# Autodesk Inventor assembly: NASA-20
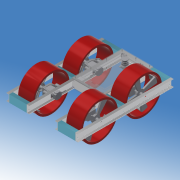
[picture p0: Inventor's stored thumbnail of the model, 180x180]
Saved by Autodesk Inventor 2020 (Build 240168000, 168)
## iProperties
RuleStatus: InUse
Created: 2019-09-05
Part Number: NASA-20
Document SubType Name: Assembly
Designer: Rick Szalay
Author: Rick Szalay
## Documents named in this file (22)
- C:\Users\mpark\Documents\NASA20\Inventor Files\NASA-20\NASA-20\NASA-20.iam
- C:\Users\mpark\Documents\NASA20\Inventor Files\NASA-20\NASA-20\A428.ipt
- C:\Users\mpark\Documents\NASA20\Inventor Files\NASA-20\NASA-20\NASA-20-WH-01.ipt
- C:\Users\mpark\Documents\NASA20\Inventor Files\NASA-20\NASA-20\NASA-20-WT-01.ipt
- C:\Users\mpark\Documents\NASA20\Inventor Files\NASA-20\NASA-20\FR\NASA-20-FR.iam
- C:\Users\mpark\Documents\NASA20\Inventor Files\NASA-20\NASA-20\FR\NASA-20-TB-01.ipt
- C:\Users\mpark\Documents\NASA20\Inventor Files\NASA-20\NASA-20\FR\NASA-20-OP-01.ipt
- C:\Users\mpark\Documents\NASA20\Inventor Files\NASA-20\NASA-20\FR\NASA-20-MP-01.ipt
- C:\Users\Matt\Documents\Inventor\Content Center Files\R2020\en-US\ANSI B18.2.1(3)\ANSI B18.2.1 - 1_4-20 UNC - 5.5(3).ipt
- C:\Users\Matt\Documents\Inventor\Content Center Files\R2020\en-US\ANSI B18.2.2(09)\ANSI B18.2.2 - 1_4 - 20(2).ipt
- C:\Users\mpark\Documents\NASA20\Inventor Files\NASA-20\NASA-20\Tube Replacements.iam
- C:\Users\mpark\Documents\NASA20\Inventor Files\NASA-20\NASA-20\E-Box\NASA-20-EBOX-B-01.ipt
- NASA-20-EBOX-B-01.ipt
- C:\Users\mpark\Documents\NASA20\Inventor Files\NASA-20\NASA-20\E-Box\NASA-20-EBOX-T-01.ipt
- NASA-20-EBOX-T-01.ipt
- C:\Users\mpark\Documents\NASA20\Inventor Files\NASA-20\NASA-20\E-Box\NASA-20-EBOX-T2-01.ipt
- C:\Users\mpark\Documents\NASA20\Inventor Files\NASA-20\NASA-20\E-Box\NASA-20-EBOX-LID-01.ipt
- C:\Users\mpark\Documents\NASA20\Inventor Files\NASA-20\NASA-20\E-Box\1603A230_UNFINISHED BRASS SURFACE-MNT HINGE W HOLES.ipt
- C:\Users\mpark\OneDrive\Documents\Inventor\Content Center Files\R2020\en-US\ANSI B18.2.4.2M\ANSI B18.2.4.2M - M3x0.5 - 5.5.ipt
- C:\Users\mpark\OneDrive\Documents\Inventor\Content Center Files\R2020\en-US\AS 1420\AS 1420 - 1973 - M3 x 14.ipt
- C:\Users\mpark\OneDrive\Documents\Inventor\Content Center Files\R2020\en-US\AS 1420\AS 1420 - 1973 - M3 x 16.ipt
- C:\Users\mpark\Documents\NASA20\Inventor Files\NASA-20\NASA-20\E-Box\9235K200_METAL 30 MM PANEL-MOUNT SWITCH.ipt
## Components (104 placed, 19 different names)
1. A428:1 — Mate:38, Mate:39, Flush:28, Mate:41
2. NASA-20-WH-01:1 — Mate:6, Flush:9, Mate:40, Mate:41
3. NASA-20-WT-01:1 — Mate:6, Flush:9, Mate:61, Tangent:1
4. NASA-20-FR:1 [sub-assembly] — Mate:20, Mate:21, Flush:13, Mate:22, Mate:23, Mate:24, Mate:25, Mate:26, Mate:27, Mate:28, Mate:29, Mate:30, Mate:31, Mate:32, Mate:33, Mate:34, Mate:35, Flush:26, Flush:27, Flush:29, Mate:42, Mate:58, Flush:36, Mate:59, Mate:60, Flush:37, Flush:38, Insert:13, Insert:14, Insert:15, Insert:16, Insert:17, Insert:18, Insert:19, Insert:20, Insert:21, Insert:22, Insert:23, Insert:24, Mate:64, Mate:65, Mate:66, Mate:67, Mate:68, Mate:69, Mate:70, Mate:71, Mate:72, Mate:73, Mate:74, Mate:75, Mate:76, Mate:77, Mate:78, Mate:79, Mate:80, Mate:81, Mate:82, Mate:83, Flush:39, Flush:40, Flush:41, Flush:42, Flush:51
5. NASA-20-OP-01:1 — Flush:24, Flush:25, Mate:37, Flush:26, Flush:27, Mate:63, Insert:7, Insert:8, Insert:9, Insert:10, Insert:11, Insert:12
6. NASA-20-OP-01:2 — Flush:24, Flush:25, Mate:36, Insert:1, Insert:2, Insert:3, Insert:4, Insert:5, Insert:6
7. NASA-20-MP-01:1 — Mate:38, Mate:39, Flush:28, Mate:40, Flush:29, Mate:42
8. A428:2
9. NASA-20-WH-01:2
10. NASA-20-WT-01:2 — Mate:62, Tangent:1
11. NASA-20-MP-01:2 — Mate:58, Flush:36
12. A428:3
13. NASA-20-WH-01:3
14. NASA-20-WT-01:3 — Mate:62, Mate:63
15. NASA-20-MP-01:3 — Mate:59, Flush:37
16. A428:4
17. NASA-20-WH-01:4
18. NASA-20-WT-01:4 — Mate:61
19. NASA-20-MP-01:4 — Mate:60, Flush:38
20. 9235K200_METAL 30 MM PANEL-MOUNT SWITCH:1
21. NASA-20-TB-01:1 — Flush:14, Mate:22, Mate:23
22. NASA-20-TB-01:2 — Flush:14, Flush:15, Mate:24, Mate:36
23. NASA-20-TB-01:3 — Flush:15, Flush:16, Mate:25
24. NASA-20-TB-01:4 — Flush:16, Flush:17, Mate:26
25. NASA-20-TB-01:5 — Flush:17, Flush:18, Mate:27
26. NASA-20-TB-01:6 — Flush:18, Mate:28
27. NASA-20-TB-01:7 — Mate:34, Mate:37
28. NASA-20-TB-01:8 — Mate:35
29. NASA-20-TB-01:9 — Mate:30
30. NASA-20-TB-01:10 — Mate:33
31. NASA-20-TB-01:11 — Mate:32
32. NASA-20-TB-01:12 — Mate:29, Mate:31
33. AS 1420 - Metric M3 x 16:11 — Insert:39
34. AS 1420 - Metric M3 x 16:12 — Insert:40
35. AS 1420 - Metric M3 x 16:13 — Insert:41
36. AS 1420 - Metric M3 x 16:14 — Insert:42
37. AS 1420 - Metric M3 x 16:15 — Insert:43
38. AS 1420 - Metric M3 x 16:16 — Insert:44
39. AS 1420 - Metric M3 x 16:17 — Insert:45
40. AS 1420 - Metric M3 x 16:18 — Insert:46
41. AS 1420 - Metric M3 x 16:19 — Insert:47
42. AS 1420 - Metric M3 x 16:20 — Insert:48
43. AS 1420 - Metric M3 x 16:1 — Insert:29
44. AS 1420 - Metric M3 x 16:2 — Insert:30
45. AS 1420 - Metric M3 x 16:3 — Insert:31
46. AS 1420 - Metric M3 x 16:4 — Insert:32
47. AS 1420 - Metric M3 x 16:5 — Insert:33
48. AS 1420 - Metric M3 x 16:6 — Insert:34
49. AS 1420 - Metric M3 x 16:7 — Insert:35
50. AS 1420 - Metric M3 x 16:8 — Insert:36
51. AS 1420 - Metric M3 x 16:9 — Insert:37
52. AS 1420 - Metric M3 x 16:10 — Insert:38
53. ANSI B18.2.4.2M M3x0.5:3 — Mate:104, Mate:106
54. ANSI B18.2.4.2M M3x0.5:4 — Mate:107, Mate:108
55. ANSI B18.2.4.2M M3x0.5:5 — Mate:109, Mate:110
56. ANSI B18.2.4.2M M3x0.5:6 — Mate:111, Mate:112
57. ANSI B18.2.4.2M M3x0.5:7 — Mate:113, Mate:114
58. ANSI B18.2.4.2M M3x0.5:8 — Mate:115, Mate:116
59. ANSI B18.2.4.2M M3x0.5:9 — Mate:117, Mate:118
60. AS 1420 - Metric M3 x 14:5 — Mate:98, Mate:99, Mate:117
61. AS 1420 - Metric M3 x 14:6 — Mate:100, Mate:101, Mate:115
62. AS 1420 - Metric M3 x 14:7 — Insert:27, Mate:111
63. AS 1420 - Metric M3 x 14:8 — Insert:28, Mate:113
64. AS 1420 - Metric M3 x 14:1 — Insert:25, Mate:109
65. AS 1420 - Metric M3 x 14:2 — Insert:26, Mate:97
66. AS 1420 - Metric M3 x 14:3 — Mate:92, Mate:96, Mate:107
67. AS 1420 - Metric M3 x 14:4 — Mate:94, Mate:95, Mate:104
68. ANSI B18.2.4.2M M3x0.5:1 — Mate:97, Mate:105
69. Hex Cap Screw - Inch 1/4-20 UNC - 5.5:13 — Insert:1
70. Hex Cap Screw - Inch 1/4-20 UNC - 5.5:14 — Insert:2
71. Hex Cap Screw - Inch 1/4-20 UNC - 5.5:15 — Insert:3
72. Hex Cap Screw - Inch 1/4-20 UNC - 5.5:16 — Insert:4
73. Hex Cap Screw - Inch 1/4-20 UNC - 5.5:17 — Insert:5
74. Hex Cap Screw - Inch 1/4-20 UNC - 5.5:18 — Insert:6
75. Hex Cap Screw - Inch 1/4-20 UNC - 5.5:20 — Insert:7
76. Hex Cap Screw - Inch 1/4-20 UNC - 5.5:19 — Insert:8
77. Hex Cap Screw - Inch 1/4-20 UNC - 5.5:21 — Insert:9
78. Hex Cap Screw - Inch 1/4-20 UNC - 5.5:22 — Insert:10
79. Hex Cap Screw - Inch 1/4-20 UNC - 5.5:23 — Insert:11
80. Hex Cap Screw - Inch 1/4-20 UNC - 5.5:24 — Insert:12
81. Hex Nut - Inch 1/4 - 20:13 — Insert:13
82. Hex Nut - Inch 1/4 - 20:14 — Insert:14
83. Hex Nut - Inch 1/4 - 20:15 — Insert:15
84. Hex Nut - Inch 1/4 - 20:16 — Insert:16
85. Hex Nut - Inch 1/4 - 20:17 — Insert:17
86. Hex Nut - Inch 1/4 - 20:18 — Insert:18
87. Hex Nut - Inch 1/4 - 20:19 — Insert:19
88. Hex Nut - Inch 1/4 - 20:20 — Insert:20
89. Hex Nut - Inch 1/4 - 20:21 — Insert:21
90. Hex Nut - Inch 1/4 - 20:22 — Insert:22
91. Hex Nut - Inch 1/4 - 20:23 — Insert:23
92. Hex Nut - Inch 1/4 - 20:24 — Insert:24
93. Tube Replacements:1 [sub-assembly] — Mate:64, Mate:70, Mate:81
94. Tube Replacements:2 [sub-assembly] — Mate:65, Mate:72, Mate:80
95. Tube Replacements:3 [sub-assembly] — Mate:66, Mate:71, Mate:79
96. Tube Replacements:4 [sub-assembly] — Mate:69, Mate:75, Mate:76
97. Tube Replacements:5 [sub-assembly] — Mate:68, Mate:74, Mate:77
98. Tube Replacements:6 [sub-assembly] — Mate:67, Mate:73, Mate:78
99. 1603A230_UNFINISHED BRASS SURFACE-MNT HINGE W HOLES:1 — Mate:90, Flush:49, Insert:25, Insert:26, Mate:92, Mate:94, Mate:95, Mate:96, Flush:50, Flush:51
100. 1603A230_UNFINISHED BRASS SURFACE-MNT HINGE W HOLES:2 — Mate:91, Flush:48, Mate:98, Mate:99, Mate:100, Mate:101, Insert:27, Insert:28, Flush:50
101. NASA-20-EBOX-LID-01:1 — Mate:85, Flush:45, Mate:86, Mate:87
102. NASA-20-EBOX-T2-01:2 — Mate:84, Flush:43, Flush:44, Flush:45, Mate:86, Mate:87, Mate:90, Mate:91, Flush:48, Flush:49, Insert:29, Insert:30, Insert:31, Insert:32, Insert:33, Insert:34, Insert:35, Insert:36, Insert:37, Insert:38
103. NASA-20-EBOX-T-01:1 — Mate:83, Flush:41, Flush:42, Mate:84, Flush:43, Flush:44, Mate:85, Mate:105, Mate:106, Mate:108, Mate:110, Mate:112, Mate:114, Mate:116, Mate:118
104. NASA-20-EBOX-B-01:1 — Mate:82, Flush:39, Flush:40, Insert:39, Insert:40, Insert:41, Insert:42, Insert:43, Insert:44, Insert:45, Insert:46, Insert:47, Insert:48
## Relationships (182: Mate 95, Insert 48, Flush 38, Tangent 1)
- Mate:6: NASA-20-WH-01:1 ↔ NASA-20-WT-01:1
- Flush:9 (19.05 mm): NASA-20-WH-01:1 ↔ NASA-20-WT-01:1
- Mate:20: NASA-20-FR:1
- Mate:21: NASA-20-FR:1
- Flush:13: NASA-20-FR:1
- Flush:14: NASA-20-TB-01:1 ↔ NASA-20-TB-01:2
- Flush:15: NASA-20-TB-01:2 ↔ NASA-20-TB-01:3
- Flush:16: NASA-20-TB-01:3 ↔ NASA-20-TB-01:4
- Flush:17: NASA-20-TB-01:4 ↔ NASA-20-TB-01:5
- Flush:18: NASA-20-TB-01:5 ↔ NASA-20-TB-01:6
- Mate:22: NASA-20-FR:1 ↔ NASA-20-TB-01:1
- Mate:23: NASA-20-FR:1 ↔ NASA-20-TB-01:1
- Mate:24: NASA-20-FR:1 ↔ NASA-20-TB-01:2
- Mate:25: NASA-20-FR:1 ↔ NASA-20-TB-01:3
- Mate:26: NASA-20-FR:1 ↔ NASA-20-TB-01:4
- Mate:27: NASA-20-FR:1 ↔ NASA-20-TB-01:5
- Mate:28: NASA-20-FR:1 ↔ NASA-20-TB-01:6
- [Flush]: NASA-20-TB-01:7 ↔ NASA-20-TB-01:8
- [Flush]: NASA-20-TB-01:8 ↔ NASA-20-TB-01:9
- [Flush]: NASA-20-TB-01:9 ↔ NASA-20-TB-01:10
- [Flush]: NASA-20-TB-01:10 ↔ NASA-20-TB-01:11
- [Flush]: NASA-20-TB-01:11 ↔ NASA-20-TB-01:12
- Mate:29: NASA-20-FR:1 ↔ NASA-20-TB-01:12
- Mate:30: NASA-20-FR:1 ↔ NASA-20-TB-01:9
- Mate:31: NASA-20-FR:1 ↔ NASA-20-TB-01:12
- Mate:32: NASA-20-FR:1 ↔ NASA-20-TB-01:11
- Mate:33: NASA-20-FR:1 ↔ NASA-20-TB-01:10
- Mate:34: NASA-20-FR:1 ↔ NASA-20-TB-01:7
- Mate:35: NASA-20-FR:1 ↔ NASA-20-TB-01:8
- Flush:24: NASA-20-OP-01:1 ↔ NASA-20-OP-01:2
- Flush:25: NASA-20-OP-01:1 ↔ NASA-20-OP-01:2
- Mate:36: NASA-20-OP-01:2 ↔ NASA-20-TB-01:2
- Mate:37: NASA-20-OP-01:1 ↔ NASA-20-TB-01:7
- Flush:26: NASA-20-FR:1 ↔ NASA-20-OP-01:1
- Flush:27: NASA-20-FR:1 ↔ NASA-20-OP-01:1
- Mate:38: A428:1 ↔ NASA-20-MP-01:1
- Mate:39: A428:1 ↔ NASA-20-MP-01:1
- Flush:28: A428:1 ↔ NASA-20-MP-01:1
- Mate:40 (1.5875 mm): NASA-20-WH-01:1 ↔ NASA-20-MP-01:1
- Mate:41: A428:1 ↔ NASA-20-WH-01:1
- Flush:29: NASA-20-FR:1 ↔ NASA-20-MP-01:1
- Mate:42: NASA-20-FR:1 ↔ NASA-20-MP-01:1
- [Mate]: NASA-20-WH-01:2 ↔ NASA-20-WT-01:2
- [Flush] (19.05 mm): NASA-20-WH-01:2 ↔ NASA-20-WT-01:2
- [Mate]: A428:2 ↔ NASA-20-MP-01:2
- [Mate]: A428:2 ↔ NASA-20-MP-01:2
- [Flush]: A428:2 ↔ NASA-20-MP-01:2
- [Mate] (1.5875 mm): NASA-20-WH-01:2 ↔ NASA-20-MP-01:2
- [Mate]: A428:2 ↔ NASA-20-WH-01:2
- [Mate]: NASA-20-WH-01:3 ↔ NASA-20-WT-01:3
- [Flush] (19.05 mm): NASA-20-WH-01:3 ↔ NASA-20-WT-01:3
- [Mate]: A428:3 ↔ NASA-20-MP-01:3
- [Mate]: A428:3 ↔ NASA-20-MP-01:3
- [Flush]: A428:3 ↔ NASA-20-MP-01:3
- [Mate] (1.5875 mm): NASA-20-WH-01:3 ↔ NASA-20-MP-01:3
- [Mate]: A428:3 ↔ NASA-20-WH-01:3
- [Mate]: NASA-20-WH-01:4 ↔ NASA-20-WT-01:4
- [Flush] (19.05 mm): NASA-20-WH-01:4 ↔ NASA-20-WT-01:4
- [Mate]: A428:4 ↔ NASA-20-MP-01:4
- [Mate]: A428:4 ↔ NASA-20-MP-01:4
- [Flush]: A428:4 ↔ NASA-20-MP-01:4
- [Mate] (1.5875 mm): NASA-20-WH-01:4 ↔ NASA-20-MP-01:4
- [Mate]: A428:4 ↔ NASA-20-WH-01:4
- Mate:58: NASA-20-FR:1 ↔ NASA-20-MP-01:2
- Flush:36: NASA-20-FR:1 ↔ NASA-20-MP-01:2
- Mate:59: NASA-20-FR:1 ↔ NASA-20-MP-01:3
- Mate:60: NASA-20-FR:1 ↔ NASA-20-MP-01:4
- Flush:37: NASA-20-FR:1 ↔ NASA-20-MP-01:3
- Flush:38: NASA-20-FR:1 ↔ NASA-20-MP-01:4
- Mate:61: NASA-20-WT-01:1 ↔ NASA-20-WT-01:4
- Mate:62: NASA-20-WT-01:2 ↔ NASA-20-WT-01:3
- Tangent:1 (50.8 mm): NASA-20-WT-01:1 ↔ NASA-20-WT-01:2
- Mate:63: NASA-20-OP-01:1 ↔ NASA-20-WT-01:3
- Insert:1: NASA-20-OP-01:2 ↔ Hex Cap Screw - Inch 1/4-20 UNC - 5.5:13
- Insert:2: NASA-20-OP-01:2 ↔ Hex Cap Screw - Inch 1/4-20 UNC - 5.5:14
- Insert:3: NASA-20-OP-01:2 ↔ Hex Cap Screw - Inch 1/4-20 UNC - 5.5:15
- Insert:4: NASA-20-OP-01:2 ↔ Hex Cap Screw - Inch 1/4-20 UNC - 5.5:16
- Insert:5: NASA-20-OP-01:2 ↔ Hex Cap Screw - Inch 1/4-20 UNC - 5.5:17
- Insert:6: NASA-20-OP-01:2 ↔ Hex Cap Screw - Inch 1/4-20 UNC - 5.5:18
- Insert:7: NASA-20-OP-01:1 ↔ Hex Cap Screw - Inch 1/4-20 UNC - 5.5:20
- Insert:8: NASA-20-OP-01:1 ↔ Hex Cap Screw - Inch 1/4-20 UNC - 5.5:19
- Insert:9: NASA-20-OP-01:1 ↔ Hex Cap Screw - Inch 1/4-20 UNC - 5.5:21
- Insert:10: NASA-20-OP-01:1 ↔ Hex Cap Screw - Inch 1/4-20 UNC - 5.5:22
- Insert:11: NASA-20-OP-01:1 ↔ Hex Cap Screw - Inch 1/4-20 UNC - 5.5:23
- Insert:12: NASA-20-OP-01:1 ↔ Hex Cap Screw - Inch 1/4-20 UNC - 5.5:24
- Insert:13: NASA-20-FR:1 ↔ Hex Nut - Inch 1/4 - 20:13
- Insert:14: NASA-20-FR:1 ↔ Hex Nut - Inch 1/4 - 20:14
- Insert:15: NASA-20-FR:1 ↔ Hex Nut - Inch 1/4 - 20:15
- Insert:16: NASA-20-FR:1 ↔ Hex Nut - Inch 1/4 - 20:16
- Insert:17: NASA-20-FR:1 ↔ Hex Nut - Inch 1/4 - 20:17
- Insert:18: NASA-20-FR:1 ↔ Hex Nut - Inch 1/4 - 20:18
- Insert:19: NASA-20-FR:1 ↔ Hex Nut - Inch 1/4 - 20:19
- Insert:20: NASA-20-FR:1 ↔ Hex Nut - Inch 1/4 - 20:20
- Insert:21: NASA-20-FR:1 ↔ Hex Nut - Inch 1/4 - 20:21
- Insert:22: NASA-20-FR:1 ↔ Hex Nut - Inch 1/4 - 20:22
- Insert:23: NASA-20-FR:1 ↔ Hex Nut - Inch 1/4 - 20:23
- Insert:24: NASA-20-FR:1 ↔ Hex Nut - Inch 1/4 - 20:24
- Mate:64: NASA-20-FR:1 ↔ Tube Replacements:1
- Mate:65: NASA-20-FR:1 ↔ Tube Replacements:2
- Mate:66: NASA-20-FR:1 ↔ Tube Replacements:3
- Mate:67: NASA-20-FR:1 ↔ Tube Replacements:6
- Mate:68: NASA-20-FR:1 ↔ Tube Replacements:5
- Mate:69: NASA-20-FR:1 ↔ Tube Replacements:4
- Mate:70: NASA-20-FR:1 ↔ Tube Replacements:1
- Mate:71: NASA-20-FR:1 ↔ Tube Replacements:3
- Mate:72: NASA-20-FR:1 ↔ Tube Replacements:2
- Mate:73: NASA-20-FR:1 ↔ Tube Replacements:6
- Mate:74: NASA-20-FR:1 ↔ Tube Replacements:5
- Mate:75: NASA-20-FR:1 ↔ Tube Replacements:4
- Mate:76: NASA-20-FR:1 ↔ Tube Replacements:4
- Mate:77: NASA-20-FR:1 ↔ Tube Replacements:5
- Mate:78: NASA-20-FR:1 ↔ Tube Replacements:6
- Mate:79: NASA-20-FR:1 ↔ Tube Replacements:3
- Mate:80: NASA-20-FR:1 ↔ Tube Replacements:2
- Mate:81: NASA-20-FR:1 ↔ Tube Replacements:1
- Mate:82: NASA-20-FR:1 ↔ NASA-20-EBOX-B-01:1
- Mate:83: NASA-20-FR:1 ↔ NASA-20-EBOX-T-01:1
- Flush:39: NASA-20-FR:1 ↔ NASA-20-EBOX-B-01:1
- Flush:40: NASA-20-FR:1 ↔ NASA-20-EBOX-B-01:1
- Flush:41: NASA-20-FR:1 ↔ NASA-20-EBOX-T-01:1
- Flush:42: NASA-20-FR:1 ↔ NASA-20-EBOX-T-01:1
- Mate:84: NASA-20-EBOX-T2-01:2 ↔ NASA-20-EBOX-T-01:1
- Flush:43: NASA-20-EBOX-T2-01:2 ↔ NASA-20-EBOX-T-01:1
- Flush:44: NASA-20-EBOX-T2-01:2 ↔ NASA-20-EBOX-T-01:1
- Mate:85: NASA-20-EBOX-LID-01:1 ↔ NASA-20-EBOX-T-01:1
- Flush:45: NASA-20-EBOX-LID-01:1 ↔ NASA-20-EBOX-T2-01:2
- Mate:86 (1 mm): NASA-20-EBOX-LID-01:1 ↔ NASA-20-EBOX-T2-01:2
- Mate:87 (1 mm): NASA-20-EBOX-LID-01:1 ↔ NASA-20-EBOX-T2-01:2
- Mate:90: 1603A230_UNFINISHED BRASS SURFACE-MNT HINGE W HOLES:1 ↔ NASA-20-EBOX-T2-01:2
- Mate:91: 1603A230_UNFINISHED BRASS SURFACE-MNT HINGE W HOLES:2 ↔ NASA-20-EBOX-T2-01:2
- Flush:48 (38.1 mm): 1603A230_UNFINISHED BRASS SURFACE-MNT HINGE W HOLES:2 ↔ NASA-20-EBOX-T2-01:2
- Flush:49 (38.1 mm): 1603A230_UNFINISHED BRASS SURFACE-MNT HINGE W HOLES:1 ↔ NASA-20-EBOX-T2-01:2
- Insert:25: AS 1420 - Metric M3 x 14:1 ↔ 1603A230_UNFINISHED BRASS SURFACE-MNT HINGE W HOLES:1
- Insert:26: AS 1420 - Metric M3 x 14:2 ↔ 1603A230_UNFINISHED BRASS SURFACE-MNT HINGE W HOLES:1
- Mate:92: AS 1420 - Metric M3 x 14:3 ↔ 1603A230_UNFINISHED BRASS SURFACE-MNT HINGE W HOLES:1
- Mate:94: AS 1420 - Metric M3 x 14:4 ↔ 1603A230_UNFINISHED BRASS SURFACE-MNT HINGE W HOLES:1
- Mate:95: AS 1420 - Metric M3 x 14:4 ↔ 1603A230_UNFINISHED BRASS SURFACE-MNT HINGE W HOLES:1
- Mate:96: AS 1420 - Metric M3 x 14:3 ↔ 1603A230_UNFINISHED BRASS SURFACE-MNT HINGE W HOLES:1
- Mate:97: AS 1420 - Metric M3 x 14:2 ↔ ANSI B18.2.4.2M M3x0.5:1
- Mate:98: AS 1420 - Metric M3 x 14:5 ↔ 1603A230_UNFINISHED BRASS SURFACE-MNT HINGE W HOLES:2
- Mate:99: AS 1420 - Metric M3 x 14:5 ↔ 1603A230_UNFINISHED BRASS SURFACE-MNT HINGE W HOLES:2
- Mate:100: AS 1420 - Metric M3 x 14:6 ↔ 1603A230_UNFINISHED BRASS SURFACE-MNT HINGE W HOLES:2
- Mate:101: AS 1420 - Metric M3 x 14:6 ↔ 1603A230_UNFINISHED BRASS SURFACE-MNT HINGE W HOLES:2
- Insert:27: AS 1420 - Metric M3 x 14:7 ↔ 1603A230_UNFINISHED BRASS SURFACE-MNT HINGE W HOLES:2
- Insert:28: AS 1420 - Metric M3 x 14:8 ↔ 1603A230_UNFINISHED BRASS SURFACE-MNT HINGE W HOLES:2
- Flush:50: 1603A230_UNFINISHED BRASS SURFACE-MNT HINGE W HOLES:1 ↔ 1603A230_UNFINISHED BRASS SURFACE-MNT HINGE W HOLES:2
- Flush:51 (25.4 mm): NASA-20-FR:1 ↔ 1603A230_UNFINISHED BRASS SURFACE-MNT HINGE W HOLES:1
- Mate:104: ANSI B18.2.4.2M M3x0.5:3 ↔ AS 1420 - Metric M3 x 14:4
- Mate:105 (-3.175 mm): ANSI B18.2.4.2M M3x0.5:1 ↔ NASA-20-EBOX-T-01:1
- Mate:106: ANSI B18.2.4.2M M3x0.5:3 ↔ NASA-20-EBOX-T-01:1
- Mate:107: ANSI B18.2.4.2M M3x0.5:4 ↔ AS 1420 - Metric M3 x 14:3
- Mate:108: ANSI B18.2.4.2M M3x0.5:4 ↔ NASA-20-EBOX-T-01:1
- Mate:109: ANSI B18.2.4.2M M3x0.5:5 ↔ AS 1420 - Metric M3 x 14:1
- Mate:110: ANSI B18.2.4.2M M3x0.5:5 ↔ NASA-20-EBOX-T-01:1
- Mate:111: ANSI B18.2.4.2M M3x0.5:6 ↔ AS 1420 - Metric M3 x 14:7
- Mate:112: ANSI B18.2.4.2M M3x0.5:6 ↔ NASA-20-EBOX-T-01:1
- Mate:113: ANSI B18.2.4.2M M3x0.5:7 ↔ AS 1420 - Metric M3 x 14:8
- Mate:114: ANSI B18.2.4.2M M3x0.5:7 ↔ NASA-20-EBOX-T-01:1
- Mate:115: ANSI B18.2.4.2M M3x0.5:8 ↔ AS 1420 - Metric M3 x 14:6
- Mate:116 (-3.175 mm): ANSI B18.2.4.2M M3x0.5:8 ↔ NASA-20-EBOX-T-01:1
- Mate:117: ANSI B18.2.4.2M M3x0.5:9 ↔ AS 1420 - Metric M3 x 14:5
- Mate:118 (-3.175 mm): ANSI B18.2.4.2M M3x0.5:9 ↔ NASA-20-EBOX-T-01:1
- Insert:29: AS 1420 - Metric M3 x 16:1 ↔ NASA-20-EBOX-T2-01:2
- Insert:30: AS 1420 - Metric M3 x 16:2 ↔ NASA-20-EBOX-T2-01:2
- Insert:31: AS 1420 - Metric M3 x 16:3 ↔ NASA-20-EBOX-T2-01:2
- Insert:32: AS 1420 - Metric M3 x 16:4 ↔ NASA-20-EBOX-T2-01:2
- Insert:33: AS 1420 - Metric M3 x 16:5 ↔ NASA-20-EBOX-T2-01:2
- Insert:34: AS 1420 - Metric M3 x 16:6 ↔ NASA-20-EBOX-T2-01:2
- Insert:35: AS 1420 - Metric M3 x 16:7 ↔ NASA-20-EBOX-T2-01:2
- Insert:36: AS 1420 - Metric M3 x 16:8 ↔ NASA-20-EBOX-T2-01:2
- Insert:37: AS 1420 - Metric M3 x 16:9 ↔ NASA-20-EBOX-T2-01:2
- Insert:38: AS 1420 - Metric M3 x 16:10 ↔ NASA-20-EBOX-T2-01:2
- Insert:39: AS 1420 - Metric M3 x 16:11 ↔ NASA-20-EBOX-B-01:1
- Insert:40: AS 1420 - Metric M3 x 16:12 ↔ NASA-20-EBOX-B-01:1
- Insert:41: AS 1420 - Metric M3 x 16:13 ↔ NASA-20-EBOX-B-01:1
- Insert:42: AS 1420 - Metric M3 x 16:14 ↔ NASA-20-EBOX-B-01:1
- Insert:43: AS 1420 - Metric M3 x 16:15 ↔ NASA-20-EBOX-B-01:1
- Insert:44: AS 1420 - Metric M3 x 16:16 ↔ NASA-20-EBOX-B-01:1
- Insert:45: AS 1420 - Metric M3 x 16:17 ↔ NASA-20-EBOX-B-01:1
- Insert:46: AS 1420 - Metric M3 x 16:18 ↔ NASA-20-EBOX-B-01:1
- Insert:47: AS 1420 - Metric M3 x 16:19 ↔ NASA-20-EBOX-B-01:1
- Insert:48: AS 1420 - Metric M3 x 16:20 ↔ NASA-20-EBOX-B-01:1
## Named parameters: d53_d41 = 0 mm, d54_d42 = 0 mm, d55_d43 = 0 mm, d56_d44 = 0 mm, d57_d45 = 0 mm, d78_d71 = 0 mm, d79_d72 = 0 mm, d80_d73 = 0 mm, d81_d74 = 1.5875 mm, d82_d75 = 0 mm, d83_d14 = 0 mm, d84_d15 = 19.05 mm, d85_d71 = 0 mm, d86_d72 = 0 mm, d87_d73 = 0 mm, d88_d74 = 1.5875 mm, d89_d75 = 0 mm, d90_d14 = 0 mm, d91_d15 = 19.05 mm, d92_d71 = 0 mm, d93_d72 = 0 mm, d94_d73 = 0 mm, d95_d74 = 1.5875 mm, d96_d75 = 0 mm, d97_d14 = 0 mm, d98_d15 = 19.05 mm
